# Autodesk Inventor assembly: servo w lexan
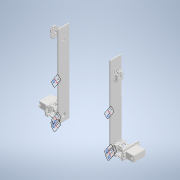
[picture p0: Inventor's stored thumbnail of the model, 180x180]
Saved by Autodesk Inventor 2020.1 (Build 241239000, 239)
## iProperties
Created: 2020-01-18
Part Number: servo w lexan
Document SubType Name: Assembly
Designer: kevin.nguyen
Author: kevin.nguyen
## Documents named in this file (6)
- C:\Users\kevin.nguyen\Desktop\Assemblies\servo w lexan.iam
- C:\Users\kevin.nguyen\Desktop\Assemblies\Servo Block.iam
- C:\Users\kevin.nguyen\Desktop\Parts Folder\615102\615102.ipt
- C:\Users\kevin.nguyen\Desktop\Parts Folder\Autodesk Made\Arm Part.ipt
- C:\Users\kevin.nguyen\Desktop\Assemblies\Sprocket w clamp.iam
- C:\Users\kevin.nguyen\Desktop\Parts Folder\535198\535198.ipt
## Components (10 placed, 5 different names)
1. Servo Block:1 [sub-assembly] — Mate:2, Mate:14
2. 615102:1 — Mate:2, Mate:7, Mate:8, Mate:9
3. Servo Block:2 [sub-assembly] — Mate:13
4. 615102:2 — Mate:10, Mate:11, Mate:12
5. Arm Part:1 — Mate:7, Mate:8, Mate:9, Mate:14, Insert:2
6. Arm Part:2 — Mate:10, Mate:11, Mate:12, Mate:13, Insert:1
7. Sprocket w clamp:1 [sub-assembly]
8. Sprocket w clamp:2 [sub-assembly]
9. 535198:1 — Insert:1
10. 535198:2 — Insert:2
## Relationships (12: Mate 10, Insert 2)
- Mate:2: Servo Block:1 ↔ 615102:1
- [Mate]: Servo Block:2 ↔ 615102:2
- Mate:7: 615102:1 ↔ Arm Part:1
- Mate:8: 615102:1 ↔ Arm Part:1
- Mate:9: 615102:1 ↔ Arm Part:1
- Mate:10: 615102:2 ↔ Arm Part:2
- Mate:11: 615102:2 ↔ Arm Part:2
- Mate:12: 615102:2 ↔ Arm Part:2
- Mate:13: Servo Block:2 ↔ Arm Part:2
- Mate:14: Servo Block:1 ↔ Arm Part:1
- Insert:1: Arm Part:2 ↔ 535198:1
- Insert:2: Arm Part:1 ↔ 535198:2
## Named parameters: d10_d1 = 0 mm
